# Autodesk Inventor assembly: conceptual assembly
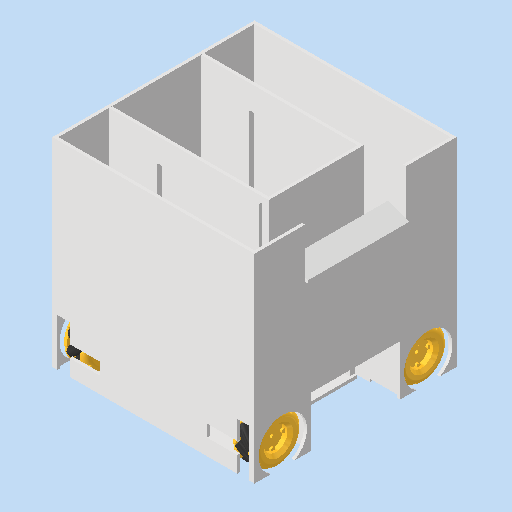
[picture p0: Inventor's stored thumbnail of the model, 512x512]
Saved by Autodesk Inventor 2026 (Build 300175000, 175)
## iProperties
Created: 2026-02-03
Part Number: conceptual assembly
Document SubType Name: Assembly
Designer: mones
Author: mones
## Documents named in this file (9)
- C:\Users\mones\OneDrive - Northeastern University\unibots\Unibots_NULondon\hardware\chassis\conceptual assembly.iam
- C:\Users\mones\OneDrive - Northeastern University\unibots\Unibots_NULondon\hardware\chassis\Chassis Conceptual Geo.ipt
- C:\Users\mones\OneDrive - Northeastern University\unibots\Unibots_NULondon\hardware\chassis\inside walls.ipt
- C:\Users\mones\OneDrive - Northeastern University\unibots\Unibots_NULondon\hardware\chassis\lift plate.ipt
- C:\Users\mones\OneDrive - Northeastern University\unibots\Unibots_NULondon\hardware\chassis\inside walls left.ipt
- C:\Users\mones\OneDrive - Northeastern University\unibots\Unibots_NULondon\hardware\chassis\inside walls front.ipt
- C:\Users\mones\OneDrive - Northeastern University\unibots\Unibots_NULondon\hardware\chassis\Mecanum Left v5\Mecanum Left.iam
- C:\Users\mones\OneDrive - Northeastern University\unibots\Unibots_NULondon\hardware\chassis\Mecanum Left v5\Mecanum Left_MIR.iam
- C:\Users\small.ab\Desktop\RoboticsGHIT\Unibots_NULondon\hardware\camera_mounts\Camera\Сборка1.iam
## Components (10 placed, 8 different names)
1. Chassis Conceptual Geo:1 — Mate:3, Mate:4, Mate:5, Mate:6, Mate:8, Insert:2, Insert:3, Insert:4, Insert:5
2. inside walls:3 — Mate:3, Mate:4, Insert:1, Mate:9
3. lift plate:1 — Insert:1
4. inside walls left:1 — Mate:5, Mate:6
5. inside walls front:1 — Mate:8, Mate:9
6. Сборка1:1 [sub-assembly]
7. Mecanum Left:1 [sub-assembly] — Insert:4
8. Mecanum Left:2 [sub-assembly] — Insert:5
9. Mecanum Left_MIR:1 [sub-assembly] — Insert:2
10. Mecanum Left_MIR:2 [sub-assembly] — Insert:3
## Relationships (11: Mate 6, Insert 5)
- Mate:3: Chassis Conceptual Geo:1 ↔ inside walls:3
- Mate:4: Chassis Conceptual Geo:1 ↔ inside walls:3
- Insert:1: inside walls:3 ↔ lift plate:1
- Mate:5: Chassis Conceptual Geo:1 ↔ inside walls left:1
- Mate:6: Chassis Conceptual Geo:1 ↔ inside walls left:1
- Mate:8: Chassis Conceptual Geo:1 ↔ inside walls front:1
- Mate:9: inside walls:3 ↔ inside walls front:1
- Insert:2 (4 mm): Chassis Conceptual Geo:1 ↔ Mecanum Left_MIR:1
- Insert:3 (4 mm): Chassis Conceptual Geo:1 ↔ Mecanum Left_MIR:2
- Insert:4 (4 mm): Chassis Conceptual Geo:1 ↔ Mecanum Left:1
- Insert:5 (4 mm): Chassis Conceptual Geo:1 ↔ Mecanum Left:2
